# Autodesk Inventor assembly: cover2
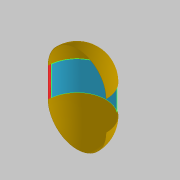
[picture p0: Inventor's stored thumbnail of the model, 180x180]
Saved by Autodesk Inventor 2021 (Build 250183000, 183)
## iProperties
Created: 2021-05-31
Part Number: cover2
Document SubType Name: Assembly
Designer: Watchdog
Author: Watchdog
## Documents named in this file (4)
- C:\Users\Watchdog\OneDrive - Flinders\Advn Mech Design Shared\6_Development\2_Design\inventor\cover\cover2.iam
- C:\Users\Watchdog\OneDrive - Flinders\Advn Mech Design Shared\6_Development\2_Design\inventor\cover\cover2_end.ipt
- C:\Users\Watchdog\OneDrive - Flinders\Advn Mech Design Shared\6_Development\2_Design\inventor\cover\cover2_shell_large.ipt
- C:\Users\Watchdog\OneDrive - Flinders\Advn Mech Design Shared\6_Development\2_Design\inventor\cover\cover2_shell_small.ipt
## Components (4 placed, 3 different names)
1. cover2_end:1 — Mate:4, Flush:6, Flush:7, Tangent:1, Mate:5, Flush:8, Mate:6
2. cover2_shell_large:1 — Tangent:1, Mate:5, Flush:8, Tangent:2, Tangent:3, Mate:7, Flush:9
3. cover2_shell_small:1 — Tangent:2, Mate:6
4. cover2_end:2 — Tangent:3, Mate:7, Flush:9
## Relationships (11: Mate 4, Flush 4, Tangent 3)
- Mate:4: cover2_end:1
- Flush:6: cover2_end:1
- Flush:7: cover2_end:1
- Tangent:1: cover2_end:1 ↔ cover2_shell_large:1
- Mate:5: cover2_end:1 ↔ cover2_shell_large:1
- Flush:8: cover2_end:1 ↔ cover2_shell_large:1
- Tangent:2: cover2_shell_large:1 ↔ cover2_shell_small:1
- Mate:6: cover2_end:1 ↔ cover2_shell_small:1
- Tangent:3: cover2_shell_large:1 ↔ cover2_end:2
- Mate:7: cover2_shell_large:1 ↔ cover2_end:2
- Flush:9: cover2_shell_large:1 ↔ cover2_end:2
